# Autodesk Inventor assembly: A2017_T4_14
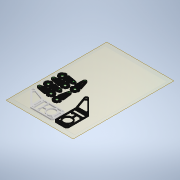
[picture p0: Inventor's stored thumbnail of the model, 180x180]
Saved by Autodesk Inventor 2020 (Build 240168000, 168)
## iProperties
Created: 2021-08-27
Part Number: A2017_T4_14
Document SubType Name: Assembly
Designer: Masato
Author: Masato
## Documents named in this file (5)
- D:\GitHub\inventor\SUSTAINA-OP\Cam\A2017_T4_14.iam
- D:\GitHub\inventor\SUSTAINA-OP\Cam\DisposableBoard.ipt
- D:\GitHub\inventor\SUSTAINA-OP\UpperBody\Trunk\Trunk_shoulder_frame.ipt
- D:\GitHub\inventor\SUSTAINA-OP\UpperBody\Trunk\Trunk_shoulder_frame_MIR.ipt
- D:\GitHub\inventor\SUSTAINA-OP\LowerBody\Ankle\Ankle_side_pitch_frame.ipt
## Components (9 placed, 4 different names)
1. DisposableBoard:1 — メイト:2, メイト:1, フラッシュ:1, フラッシュ:2, メイト:6, メイト:13, メイト:14, メイト:15, 正接:1, メイト:17, メイト:18, 正接:2, 正接:3, メイト:20, メイト:21
2. Trunk_shoulder_frame_MIR:1 — メイト:6, メイト:13, メイト:16, 正接:1, 正接:4, 正接:6
3. Trunk_shoulder_frame:1 — メイト:14, メイト:15, メイト:16
4. Ankle_side_pitch_frame:5 — メイト:20, 正接:5, 正接:6, 正接:7
5. Ankle_side_pitch_frame:6 — メイト:21, 正接:7, 正接:8, 正接:9
6. Ankle_side_pitch_frame:2 — メイト:18, メイト:19, 角度:1, 正接:2
7. Ankle_side_pitch_frame:1 — メイト:17, メイト:19, 正接:3, 正接:4, 正接:5
8. Ankle_side_pitch_frame:3 — 正接:8
9. Ankle_side_pitch_frame:4 — 正接:9
## Component patterns: (2 elements, first: Ankle_side_pitch_frame:2 + Ankle_side_pitch_frame:1)
## Relationships (24: Mate 12, Tangent 9, Flush 2, Angle 1)
- メイト:2 [Mate]: DisposableBoard:1
- メイト:1 [Mate]: DisposableBoard:1
- フラッシュ:1 [Flush]: DisposableBoard:1
- フラッシュ:2 [Flush]: DisposableBoard:1
- メイト:6 [Mate]: DisposableBoard:1 ↔ Trunk_shoulder_frame_MIR:1
- メイト:13 [Mate] (2 mm): DisposableBoard:1 ↔ Trunk_shoulder_frame_MIR:1
- メイト:14 [Mate]: DisposableBoard:1 ↔ Trunk_shoulder_frame:1
- メイト:15 [Mate] (2 mm): DisposableBoard:1 ↔ Trunk_shoulder_frame:1
- メイト:16 [Mate] (2.5 mm): Trunk_shoulder_frame_MIR:1 ↔ Trunk_shoulder_frame:1
- 正接:1 [Tangent] (2 mm): DisposableBoard:1 ↔ Trunk_shoulder_frame_MIR:1
- メイト:17 [Mate]: DisposableBoard:1 ↔ Ankle_side_pitch_frame:1
- メイト:18 [Mate]: DisposableBoard:1 ↔ Ankle_side_pitch_frame:2
- メイト:19 [Mate] (2.5 mm): Ankle_side_pitch_frame:2 ↔ Ankle_side_pitch_frame:1
- 角度:1 [Angle] (0 deg): Ankle_side_pitch_frame:2
- 正接:2 [Tangent] (3 mm): DisposableBoard:1 ↔ Ankle_side_pitch_frame:2
- 正接:3 [Tangent] (3 mm): DisposableBoard:1 ↔ Ankle_side_pitch_frame:1
- 正接:4 [Tangent] (8 mm): Trunk_shoulder_frame_MIR:1 ↔ Ankle_side_pitch_frame:1
- メイト:20 [Mate]: DisposableBoard:1 ↔ Ankle_side_pitch_frame:5
- メイト:21 [Mate]: DisposableBoard:1 ↔ Ankle_side_pitch_frame:6
- 正接:5 [Tangent] (2.5 mm): Ankle_side_pitch_frame:5 ↔ Ankle_side_pitch_frame:1
- 正接:6 [Tangent] (10 mm): Trunk_shoulder_frame_MIR:1 ↔ Ankle_side_pitch_frame:5
- 正接:7 [Tangent] (2.5 mm): Ankle_side_pitch_frame:5 ↔ Ankle_side_pitch_frame:6
- 正接:8 [Tangent] (2.5 mm): Ankle_side_pitch_frame:6 ↔ Ankle_side_pitch_frame:3
- 正接:9 [Tangent] (2.5 mm): Ankle_side_pitch_frame:6 ↔ Ankle_side_pitch_frame:4
